# Autodesk Inventor assembly: arm
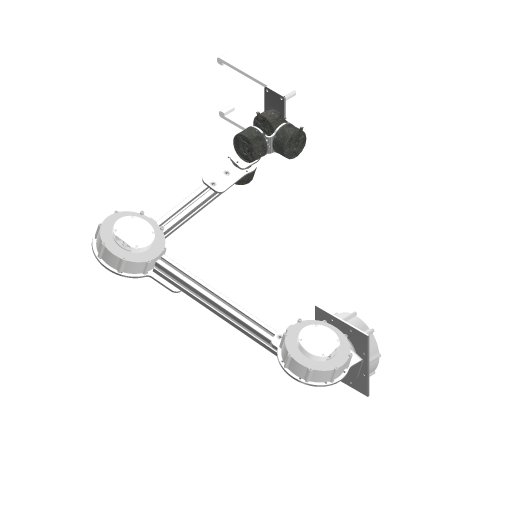
[picture p0: Inventor's stored thumbnail of the model, 512x512]
Saved by Autodesk Inventor 2024.3 (Build 283343000, 343)
## iProperties
Created: 2024-10-12
Part Number: arm
Document SubType Name: Assembly
Designer: haya
Mass: 2181.66 g
Surface Area: 3955.94 cm^2
Volume: 749.287 cm^3
Author: haya
## Documents named in this file (16)
- C:\Users\haya\Documents\GitHub\rdc_arm\arm.iam
- C:\Users\haya\Documents\GitHub\rdc_arm\base_plate.ipt
- C:\Users\haya\Documents\GitHub\rdc_arm\8108-8\8108-8.iam
- C:\Users\haya\Documents\GitHub\rdc_arm\shoulder_plate.ipt
- C:\Users\haya\Documents\GitHub\rdc_arm\link_plate.ipt
- C:\Users\haya\Documents\GitHub\rdc_arm\GIM3505-8.ipt
- C:\Users\haya\Documents\GitHub\rdc_arm\TF-M5-2.ipt
- C:\Users\haya\Documents\GitHub\rdc_arm\HFS5-2020-300-Z5-XA10-XB40-XC260-XD290.ipt
- C:\Users\haya\Documents\GitHub\rdc_arm\elbow_plate.ipt
- C:\Users\haya\Documents\GitHub\rdc_arm\wrist_pitch_plate.ipt
- C:\Users\haya\Documents\GitHub\rdc_arm\wrist_pitch_spacer.ipt
- C:\Users\haya\Documents\GitHub\rdc_arm\wrist_yaw_plate.ipt
- C:\Users\haya\Documents\GitHub\rdc_arm\hand_plate.ipt
- C:\Users\haya\Documents\GitHub\rdc_arm\finger_plate.ipt
- C:\Users\haya\Documents\GitHub\rdc_arm\finger_plastic.ipt
- C:\Users\haya\Documents\GitHub\rdc_arm\HFS5-2020-300-Z5-XA10-XB40-XC260-XD290_2.ipt
## Components (33 placed, 15 different names)
1. base_plate:1 — 挿入:1, メイト:25, 角度:8, 角度:9, メイト:29, フラッシュ:3, 角度:10, 角度:11
2. 8108-8:1 [sub-assembly] — 挿入:1, 挿入:3, 挿入:4, メイト:26, メイト:27
3. shoulder_plate:1 — 挿入:3, 挿入:4, 挿入:75, 角度:8, 角度:6
4. 8108-8:2 [sub-assembly] — 挿入:20, 挿入:21, 挿入:75
5. 8108-8:3 [sub-assembly] — 挿入:27, 挿入:28, 挿入:34
6. link_plate:1 — 挿入:20, 挿入:21, 挿入:32, 挿入:33, メイト:10, メイト:23, フラッシュ:1, 角度:6
7. link_plate:2 — 挿入:27, 挿入:28, メイト:16, メイト:17, メイト:18, 挿入:38, 挿入:39, フラッシュ:2, メイト:24, 角度:7
8. GIM3505-8:1 — 挿入:44, 挿入:45, 挿入:80
9. TF-M5-2:1 — 挿入:32
10. TF-M5-2:2 — 挿入:33
11. HFS5-2020-300-Z5-XA10-XB40-XC260-XD290:1 — メイト:10, メイト:23, フラッシュ:1, 挿入:78, 挿入:79
12. elbow_plate:1 — 挿入:34, 角度:7, 挿入:76, 挿入:77, 挿入:78, 挿入:79
13. TF-M5-2:3 — 挿入:77
14. TF-M5-2:4 — 挿入:76
15. HFS5-2020-300-Z5-XA10-XB40-XC260-XD290_2:1 — メイト:16, メイト:17, メイト:18, メイト:19, メイト:20, メイト:21, 60, フラッシュ:2, メイト:24
16. TF-M5-2:5 — 挿入:38
17. TF-M5-2:6 — 挿入:39
18. wrist_pitch_plate:1 — メイト:19, メイト:20, メイト:21, 角度:4, 挿入:80, 挿入:81, 挿入:82
19. TF-M5-2:7 — 挿入:82
20. TF-M5-2:8 — 挿入:81
21. wrist_pitch_spacer:1 — 挿入:44, 挿入:45, 挿入:69, 挿入:70
22. wrist_yaw_plate:1 — 挿入:47, 60, 挿入:69, 挿入:70
23. GIM3505-8:2 — 挿入:47, 挿入:71
24. wrist_pitch_spacer:2 — 挿入:71, 挿入:72, メイト:22
25. GIM3505-8:3 — 挿入:55, 挿入:56, 挿入:73, 挿入:74
26. wrist_pitch_spacer:3 — 挿入:55, 挿入:56, 挿入:63
27. hand_plate:1 — 挿入:59, 挿入:60, 挿入:63, 挿入:64, 挿入:65, 角度:3, 角度:5
28. GIM3505-8:4 — 挿入:59, 挿入:60, 挿入:61, 挿入:62
29. wrist_pitch_spacer:4 — 挿入:61, 挿入:62, 挿入:66
30. finger_plate:1 — 挿入:64, 挿入:65, 角度:10, 角度:11
31. finger_plastic:1 — 挿入:66, 角度:3, 挿入:67, 挿入:68
32. finger_plate:2 — 挿入:67, 挿入:68, メイト:29, フラッシュ:3
33. wrist_yaw_plate:2 — 挿入:72, メイト:22, 角度:4, 挿入:73, 挿入:74, 角度:5
## Relationships (68: Insert 41, Mate 14, Angle 10, Flush 3)
- 挿入:1 [Insert]: base_plate:1 ↔ 8108-8:1
- 挿入:3 [Insert]: 8108-8:1 ↔ shoulder_plate:1
- 挿入:4 [Insert]: 8108-8:1 ↔ shoulder_plate:1
- 挿入:20 [Insert]: 8108-8:2 ↔ link_plate:1
- 挿入:21 [Insert]: 8108-8:2 ↔ link_plate:1
- 挿入:27 [Insert]: 8108-8:3 ↔ link_plate:2
- 挿入:28 [Insert]: 8108-8:3 ↔ link_plate:2
- 挿入:32 [Insert]: link_plate:1 ↔ TF-M5-2:1
- 挿入:33 [Insert]: link_plate:1 ↔ TF-M5-2:2
- メイト:10 [Mate]: link_plate:1 ↔ HFS5-2020-300-Z5-XA10-XB40-XC260-XD290:1
- 挿入:34 [Insert]: 8108-8:3 ↔ elbow_plate:1
- メイト:16 [Mate]: link_plate:2 ↔ HFS5-2020-300-Z5-XA10-XB40-XC260-XD290_2:1
- メイト:17 [Mate]: link_plate:2 ↔ HFS5-2020-300-Z5-XA10-XB40-XC260-XD290_2:1
- メイト:18 [Mate]: link_plate:2 ↔ HFS5-2020-300-Z5-XA10-XB40-XC260-XD290_2:1
- 挿入:38 [Insert]: link_plate:2 ↔ TF-M5-2:5
- 挿入:39 [Insert]: link_plate:2 ↔ TF-M5-2:6
- メイト:19 [Mate]: HFS5-2020-300-Z5-XA10-XB40-XC260-XD290_2:1 ↔ wrist_pitch_plate:1
- メイト:20 [Mate]: HFS5-2020-300-Z5-XA10-XB40-XC260-XD290_2:1 ↔ wrist_pitch_plate:1
- メイト:21 [Mate]: HFS5-2020-300-Z5-XA10-XB40-XC260-XD290_2:1 ↔ wrist_pitch_plate:1
- 挿入:44 [Insert]: GIM3505-8:1 ↔ wrist_pitch_spacer:1
- 挿入:45 [Insert]: GIM3505-8:1 ↔ wrist_pitch_spacer:1
- 挿入:47 [Insert]: wrist_yaw_plate:1 ↔ GIM3505-8:2
- 60 [Angle] (60 deg): HFS5-2020-300-Z5-XA10-XB40-XC260-XD290_2:1 ↔ wrist_yaw_plate:1
- 挿入:55 [Insert]: GIM3505-8:3 ↔ wrist_pitch_spacer:3
- 挿入:56 [Insert]: GIM3505-8:3 ↔ wrist_pitch_spacer:3
- 挿入:59 [Insert]: hand_plate:1 ↔ GIM3505-8:4
- 挿入:60 [Insert]: hand_plate:1 ↔ GIM3505-8:4
- 挿入:61 [Insert]: GIM3505-8:4 ↔ wrist_pitch_spacer:4
- 挿入:62 [Insert]: GIM3505-8:4 ↔ wrist_pitch_spacer:4
- 挿入:63 [Insert]: wrist_pitch_spacer:3 ↔ hand_plate:1
- 挿入:64 [Insert]: hand_plate:1 ↔ finger_plate:1
- 挿入:65 [Insert]: hand_plate:1 ↔ finger_plate:1
- 挿入:66 [Insert]: wrist_pitch_spacer:4 ↔ finger_plastic:1
- 角度:3 [Angle] (180 deg): hand_plate:1 ↔ finger_plastic:1
- 挿入:67 [Insert]: finger_plastic:1 ↔ finger_plate:2
- 挿入:68 [Insert]: finger_plastic:1 ↔ finger_plate:2
- 挿入:69 [Insert]: wrist_pitch_spacer:1 ↔ wrist_yaw_plate:1
- 挿入:70 [Insert]: wrist_pitch_spacer:1 ↔ wrist_yaw_plate:1
- 挿入:71 [Insert]: GIM3505-8:2 ↔ wrist_pitch_spacer:2
- 挿入:72 [Insert]: wrist_pitch_spacer:2 ↔ wrist_yaw_plate:2
- メイト:22 [Mate]: wrist_pitch_spacer:2 ↔ wrist_yaw_plate:2
- 角度:4 [Angle] (40 deg): wrist_pitch_plate:1 ↔ wrist_yaw_plate:2
- 挿入:73 [Insert]: GIM3505-8:3 ↔ wrist_yaw_plate:2
- 挿入:74 [Insert]: GIM3505-8:3 ↔ wrist_yaw_plate:2
- 角度:5 [Angle] (0 deg): hand_plate:1 ↔ wrist_yaw_plate:2
- メイト:23 [Mate] (-47 mm): link_plate:1 ↔ HFS5-2020-300-Z5-XA10-XB40-XC260-XD290:1
- フラッシュ:1 [Flush] (8 mm): link_plate:1 ↔ HFS5-2020-300-Z5-XA10-XB40-XC260-XD290:1
- フラッシュ:2 [Flush] (8 mm): link_plate:2 ↔ HFS5-2020-300-Z5-XA10-XB40-XC260-XD290_2:1
- メイト:24 [Mate] (-47 mm): link_plate:2 ↔ HFS5-2020-300-Z5-XA10-XB40-XC260-XD290_2:1
- 挿入:75 [Insert]: shoulder_plate:1 ↔ 8108-8:2
- 角度:8 [Angle] (0 deg): base_plate:1 ↔ shoulder_plate:1
- 角度:6 [Angle] (60 deg): shoulder_plate:1 ↔ link_plate:1
- 角度:7 [Angle] (90 deg): link_plate:2 ↔ elbow_plate:1
- メイト:25 [Mate]: base_plate:1
- メイト:26 [Mate]: 8108-8:1
- メイト:27 [Mate]: 8108-8:1
- 角度:9 [Angle] (0 deg): base_plate:1
- 挿入:76 [Insert]: elbow_plate:1 ↔ TF-M5-2:4
- 挿入:77 [Insert]: elbow_plate:1 ↔ TF-M5-2:3
- 挿入:78 [Insert]: HFS5-2020-300-Z5-XA10-XB40-XC260-XD290:1 ↔ elbow_plate:1
- 挿入:79 [Insert]: HFS5-2020-300-Z5-XA10-XB40-XC260-XD290:1 ↔ elbow_plate:1
- 挿入:80 [Insert]: GIM3505-8:1 ↔ wrist_pitch_plate:1
- 挿入:81 [Insert]: wrist_pitch_plate:1 ↔ TF-M5-2:8
- 挿入:82 [Insert]: wrist_pitch_plate:1 ↔ TF-M5-2:7
- メイト:29 [Mate] (50 mm): base_plate:1 ↔ finger_plate:2
- フラッシュ:3 [Flush] (20 mm): base_plate:1 ↔ finger_plate:2
- 角度:10 [Angle] (0 deg): base_plate:1 ↔ finger_plate:1
- 角度:11 [Angle] (0 deg): base_plate:1 ↔ finger_plate:1
